# Autodesk Inventor assembly: lifter
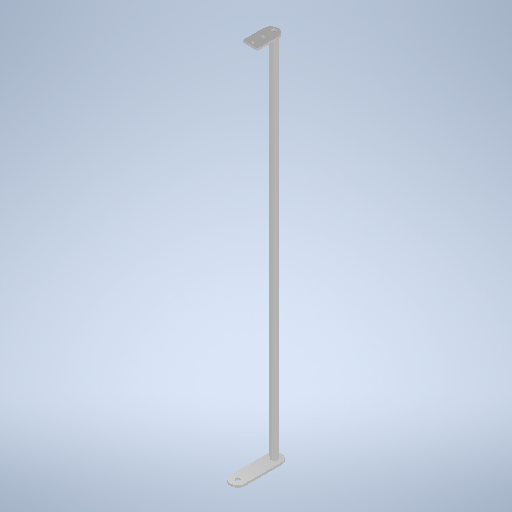
[picture p0: Inventor's stored thumbnail of the model, 512x512]
Saved by Autodesk Inventor 2025 (Build 290162000, 162)
## iProperties
Created: 2024-04-25
Part Number: lifter
Document SubType Name: Assembly
Designer: rader
Author: rader
## Documents named in this file (4)
- C:\Users\rader\Documents\rp\lifter.iam
- C:\Users\rader\Documents\rp\lifter_rod.ipt
- C:\Users\rader\Documents\rp\lifter_free_end.ipt
- C:\Users\rader\Documents\rp\lifter_servo_end.ipt
## Components (3 placed, 3 different names)
1. lifter_rod:1 — Vložit:1, Vložit:2
2. lifter_free_end:1 — Vložit:1, Stejný směr:1
3. lifter_servo_end:1 — Vložit:2, Stejný směr:1
## Relationships (3: Insert 2, Flush 1)
- Vložit:1 [Insert]: lifter_rod:1 ↔ lifter_free_end:1
- Vložit:2 [Insert]: lifter_rod:1 ↔ lifter_servo_end:1
- Stejný směr:1 [Flush]: lifter_free_end:1 ↔ lifter_servo_end:1
